# Autodesk Inventor assembly: 545340 assembly
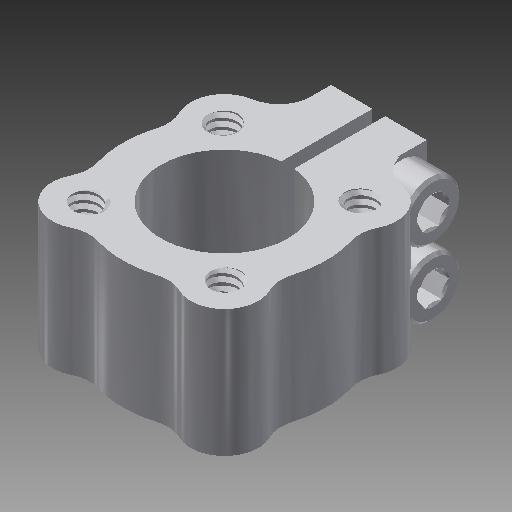
[picture p0: Inventor's stored thumbnail of the model, 512x512]
Saved by Autodesk Inventor 2017 (Build 210142000, 142)
## iProperties
Created: 2016-08-15
Part Number: 545340 assembly
Description: STEP AP203
Document SubType Name: Assembly
Designer: Dell
Mass: 3.68863 g
Surface Area: 38.6981 cm^2
Volume: 3.68863 cm^3
Density: 1 g/cm^3
Sending System: SolidWorks 2014
Preprocessor: SwSTEP 2.0
Title: 545340 assembly.STEP
Revision Number: ANY
## Documents named in this file (3)
- C:\Users\Dell\Documents\GitHub\tr2\Actuator 1.3\545340 assembly.iam
- C:\Users\Dell\Documents\GitHub\tr2\Actuator 1.3\545340.ipt
- C:\Users\Dell\Documents\GitHub\tr2\Actuator 1.3\632110_90128A121.ipt
## Components (3 placed, 3 different names)
1. 545340_1 — Mate:1, Mate:2, Mate:3, Mate:4
2. 632110_90128A121_2 — Mate:1, Mate:3
3. 632110_90128A121_3 — Mate:2, Mate:4
## Relationships (4: Mate 4)
- Mate:1: 545340_1 ↔ 632110_90128A121_2
- Mate:2: 545340_1 ↔ 632110_90128A121_3
- Mate:3: 545340_1 ↔ 632110_90128A121_2
- Mate:4: 545340_1 ↔ 632110_90128A121_3
